# Autodesk Inventor assembly: main_assembly
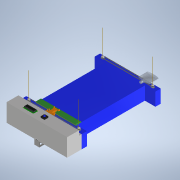
[picture p0: Inventor's stored thumbnail of the model, 180x180]
Saved by Autodesk Inventor 2020 (Build 240168000, 168)
## iProperties
Created: 2021-03-06
Part Number: main_assembly
Document SubType Name: Assembly
Designer: Harry
Author: Harry
## Documents named in this file (15)
- C:\Users\Harry\Documents\hacktheburgh\octocatch\cad\main_assembly.iam
- C:\Users\Harry\Documents\hacktheburgh\octocatch\cad\backplate.ipt
- C:\Users\Harry\Documents\hacktheburgh\octocatch\cad\dc_motor_larger.ipt
- C:\Users\Harry\Documents\hacktheburgh\octocatch\cad\belt_gear.ipt
- C:\Users\Harry\Documents\hacktheburgh\octocatch\cad\main_assembly\Design Accelerator\Synchronous Belts Transmission1.iam
- C:\Users\Harry\Documents\hacktheburgh\octocatch\cad\octopus_on_belt.ipt
- C:\Users\Harry\Documents\hacktheburgh\octocatch\cad\large_motor_with_gear.iam
- C:\Users\Harry\Documents\hacktheburgh\octocatch\cad\main_assembly\Design Accelerator\Synchronous Belts Transmission2.iam
- C:\Users\Harry\Documents\hacktheburgh\octocatch\cad\hopper assembly.iam
- C:\Users\Harry\Documents\hacktheburgh\octocatch\cad\ball_ramp.ipt
- C:\Users\Harry\Documents\hacktheburgh\octocatch\cad\ball_collector_assembly.iam
- C:\Users\Harry\Documents\hacktheburgh\octocatch\cad\marble_lift.iam
- C:\Users\Harry\Documents\hacktheburgh\octocatch\cad\tube.ipt
- C:\Users\Harry\Documents\hacktheburgh\octocatch\cad\potentiometer.iam
- C:\Users\Harry\Documents\hacktheburgh\octocatch\cad\LCD.ipt
## Components (17 placed, 13 different names)
1. backplate:1 — Insert:1, Insert:2, Insert:5, Insert:6, Mate:5, Mate:6, Mate:7, Mate:9
2. dc_motor_larger:1 — Insert:1, Insert:3
3. dc_motor_larger:2 — Insert:2, Insert:4
4. belt_gear:1 — Insert:3
5. belt_gear:2 — Insert:4
6. Synchronous Belts Transmission:1 [sub-assembly] — Mate:1, Mate:2
7. octopus_on_belt:1 — Mate:1, Mate:2
8. large_motor_with_gear:1 [sub-assembly] — Insert:5
9. large_motor_with_gear:2 [sub-assembly] — Insert:6
10. Synchronous Belts Transmission:2 [sub-assembly] — Mate:3, Mate:4
11. hopper assembly:1 [sub-assembly] — Mate:3, Mate:4, Ball:1
12. ball_ramp:1 — Mate:5
13. ball_collector_assembly:1 [sub-assembly] — Mate:6, Mate:7, Mate:8, Flush:1, Mate:11, Mate:12
14. marble_lift:1 [sub-assembly] — Mate:8, Flush:1, Mate:9, Mate:10
15. tube:1 — Ball:1, Mate:10
16. potentiometer:1 [sub-assembly] — Mate:11
17. LCD:1 — Mate:12
## Relationships (20: Mate 12, Insert 6, Flush 1, BallJoint 1)
- Insert:1: backplate:1 ↔ dc_motor_larger:1
- Insert:2: backplate:1 ↔ dc_motor_larger:2
- Insert:3: dc_motor_larger:1 ↔ belt_gear:1
- Insert:4: dc_motor_larger:2 ↔ belt_gear:2
- Mate:1: Synchronous Belts Transmission:1 ↔ octopus_on_belt:1
- Mate:2: Synchronous Belts Transmission:1 ↔ octopus_on_belt:1
- Insert:5: backplate:1 ↔ large_motor_with_gear:1
- Insert:6: backplate:1 ↔ large_motor_with_gear:2
- Mate:3: Synchronous Belts Transmission:2 ↔ hopper assembly:1
- Mate:4: Synchronous Belts Transmission:2 ↔ hopper assembly:1
- Mate:5: backplate:1 ↔ ball_ramp:1
- Mate:6: backplate:1 ↔ ball_collector_assembly:1
- Mate:7: backplate:1 ↔ ball_collector_assembly:1
- Mate:8: ball_collector_assembly:1 ↔ marble_lift:1
- Flush:1: ball_collector_assembly:1 ↔ marble_lift:1
- Mate:9 (-2.5 mm): backplate:1 ↔ marble_lift:1
- Ball:1: hopper assembly:1 ↔ tube:1
- Mate:10: marble_lift:1 ↔ tube:1
- Mate:11: ball_collector_assembly:1 ↔ potentiometer:1
- Mate:12: ball_collector_assembly:1 ↔ LCD:1
